# Autodesk Inventor assembly: short_assembly
Saved by Autodesk Inventor 2021 (Build 250183000, 183)
## iProperties
Created: 2020-12-11
Part Number: short_assembly
Document SubType Name: Assembly
Designer: Tomasz
Author: Tomasz
## Documents named in this file (3)
- T:\Dev\tco-cad\misc\short_assembly.iam
- T:\Dev\tco-cad\base_short.ipt
- T:\Dev\tco-cad\top_short.ipt
## Components (2 placed, 2 different names)
1. base_short:1 — Mate:1, Mate:2, Mate:3
2. top_short:1 — Mate:1, Mate:2, Mate:3
## Relationships (3: Mate 3)
- Mate:1 (10 mm): base_short:1 ↔ top_short:1
- Mate:2: base_short:1 ↔ top_short:1
- Mate:3: base_short:1 ↔ top_short:1
